# Autodesk Inventor assembly: speakerAssembly
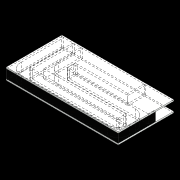
[picture p0: Inventor's stored thumbnail of the model, 180x180]
Saved by Autodesk Inventor 2022 (Build 260153000, 153)
## iProperties
Created: 2022-07-08
Part Number: speakerAssembly
Document SubType Name: Assembly
Designer: Fuzzyfish
Author: Fuzzyfish
## Documents named in this file (3)
- C:\Users\Fuzzyfish\Documents\Inventor\finalBox\speakerAssembly.iam
- C:\Users\Fuzzyfish\Documents\Inventor\finalBox\midPath.ipt
- C:\Users\Fuzzyfish\Documents\Inventor\finalBox\acrylic panel.ipt
## Components (3 placed, 2 different names)
1. midPath:1 — Flush:1, Mate:1, Flush:2, Mate:2, Flush:3, Flush:4
2. acrylic panel:1 — Flush:1, Mate:1, Flush:2
3. acrylic panel:2 — Mate:2, Flush:3, Flush:4
## Relationships (6: Flush 4, Mate 2)
- Flush:1: midPath:1 ↔ acrylic panel:1
- Mate:1: midPath:1 ↔ acrylic panel:1
- Flush:2: midPath:1 ↔ acrylic panel:1
- Mate:2: midPath:1 ↔ acrylic panel:2
- Flush:3: midPath:1 ↔ acrylic panel:2
- Flush:4: midPath:1 ↔ acrylic panel:2
